# Autodesk Inventor assembly: BES870XL Portafilter_assembled
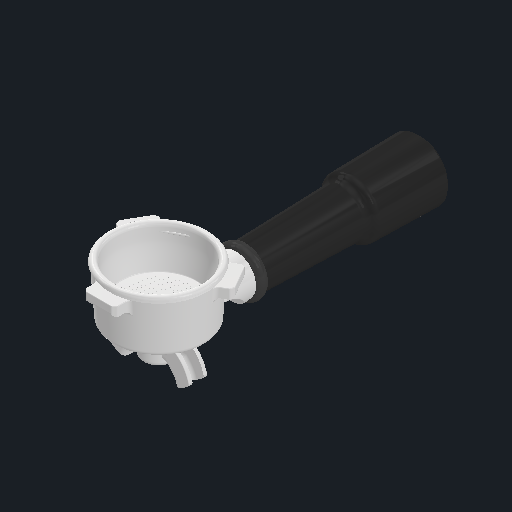
[picture p0: Inventor's stored thumbnail of the model, 512x512]
Saved by Autodesk Inventor 2026 (Build 300175000, 175)
## iProperties
Created: 2019-03-08
Part Number: BES870XL Portafilter_assembled
Document SubType Name: Assembly
Designer: Paul Juschitz
Sending System: Autodesk Translation Framework v7.6.0.251
Preprocessor: ST-DEVELOPER v17.2
Title: D:/grabcad/bes870xl-portafilter/BES870XL Portafilter.step
Author: vincebshock
## Documents named in this file (4)
- C:\Users\Paul Juschitz\Documents\private\m5_GBW_mod\M5_GBW_mod\CAD\downloads\portafilter\BES870XL Portafilter\BES870XL Portafilter\BES870XL Portafilter_assembled.iam
- C:\Users\Paul Juschitz\Documents\private\m5_GBW_mod\M5_GBW_mod\CAD\downloads\portafilter\BES870XL Portafilter\BES870XL Portafilter\portafilter.iam
- C:\Users\Paul Juschitz\Documents\private\m5_GBW_mod\M5_GBW_mod\CAD\downloads\portafilter\BES870XL Portafilter\BES870XL Portafilter\double shot basket.ipt
- C:\Users\Paul Juschitz\Documents\private\m5_GBW_mod\M5_GBW_mod\CAD\downloads\portafilter\BES870XL Portafilter\BES870XL Portafilter\double-spout.ipt
## Components (3 placed, 3 different names)
1. portafilter:1 [sub-assembly] — Cylindrical:1, Cylindrical:2, Angle:1
2. double shot basket:1 — Cylindrical:1
3. double-spout:1 — Cylindrical:2, Angle:1
## Relationships (3: CylindricalJoint 2, Angle 1)
- Cylindrical:1: portafilter:1 ↔ double shot basket:1
- Cylindrical:2: portafilter:1 ↔ double-spout:1
- Angle:1 (0 deg): portafilter:1 ↔ double-spout:1
